# Autodesk Inventor assembly: Assembly2
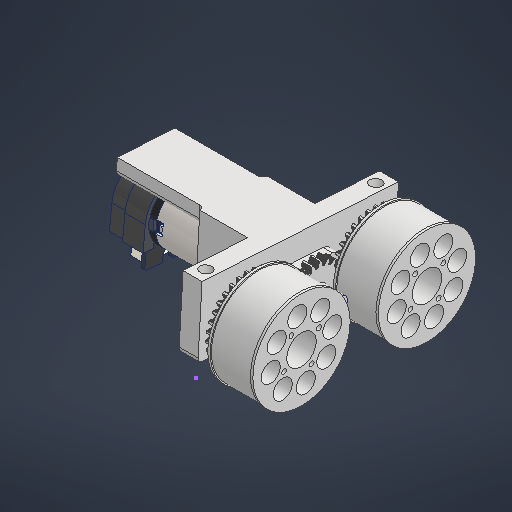
[picture p0: Inventor's stored thumbnail of the model, 512x512]
Saved by Autodesk Inventor 2027 (Build 310192060, 192F)
## iProperties
Created: 2026-08-12
Part Number: Assembly2
Document SubType Name: Assembly
Designer: felip
Author: felip
## Documents named in this file (6)
- C:\Users\felip\OneDrive\Escritorio\Laberinto2026\GCM\GCMV1\GCMPlaca\CAD\Assembly2.iam
- C:\Users\felip\OneDrive\Documents\mmgm-cb-enc-side-con\mmgm-cb-enc-side-con.ipt
- C:\Users\felip\OneDrive\Escritorio\Laberinto2026\GCM\GCMV1\GCMPlaca\CAD\Engranajes\EngranajeRuedaV2\EngranajeRuedaV2.ipt
- C:\Users\felip\OneDrive\Escritorio\Laberinto2026\GCM\GCMV1\GCMPlaca\CAD\Modelos\PololuMount\PololuMount.ipt
- C:\Users\felip\OneDrive\Escritorio\Laberinto2026\GCM\GCMV1\GCMPlaca\CAD\Ruedas\RimV1\RimV1.ipt
- C:\Users\felip\Downloads\EngranajeMotor 2mm.ipt
## Components (7 placed, 5 different names)
1. mmgm-cb-enc-side-con:1 — Mate:1, Mate:2, Mate:7
2. PololuMount:1 — Mate:1, Mate:2, Mate:3, Mate:4, Mate:5, Mate:6, Mate:8
3. EngranajeRuedaV2:3 — Mate:3, Mate:4, Rotation:1, Mate:9, Mate:10, Mate:13
4. EngranajeRuedaV2:4 — Mate:5, Mate:6, Rotation:1, Rotation:2, Mate:11, Mate:12, Mate:14
5. RimV1:3 — Mate:9, Mate:10, Mate:13
6. RimV1:4 — Mate:11, Mate:12, Mate:14
7. EngranajeMotor 2mm:2 — Mate:7, Mate:8, Rotation:2
## Relationships (16: Mate 14, RelateRotation 2)
- Mate:1: mmgm-cb-enc-side-con:1 ↔ PololuMount:1
- Mate:2: mmgm-cb-enc-side-con:1 ↔ PololuMount:1
- Mate:3: PololuMount:1 ↔ EngranajeRuedaV2:3
- Mate:4 (0.5 mm): PololuMount:1 ↔ EngranajeRuedaV2:3
- Mate:5: PololuMount:1 ↔ EngranajeRuedaV2:4
- Mate:6 (0.5 mm): PololuMount:1 ↔ EngranajeRuedaV2:4
- Mate:7: mmgm-cb-enc-side-con:1 ↔ EngranajeMotor 2mm:2
- Mate:8 (0.5 mm): PololuMount:1 ↔ EngranajeMotor 2mm:2
- Rotation:1 [RelateRotation] (1 ul): EngranajeRuedaV2:3 ↔ EngranajeRuedaV2:4
- Rotation:2 [RelateRotation] (2.5 ul): EngranajeRuedaV2:4 ↔ EngranajeMotor 2mm:2
- Mate:9: EngranajeRuedaV2:3 ↔ RimV1:3
- Mate:10: EngranajeRuedaV2:3 ↔ RimV1:3
- Mate:11: EngranajeRuedaV2:4 ↔ RimV1:4
- Mate:12: EngranajeRuedaV2:4 ↔ RimV1:4
- Mate:13: EngranajeRuedaV2:3 ↔ RimV1:3
- Mate:14: EngranajeRuedaV2:4 ↔ RimV1:4
